# Autodesk Inventor assembly: acrylic kinect bracket - manufacturing
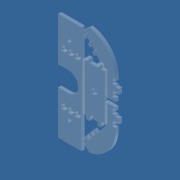
[picture p0: Inventor's stored thumbnail of the model, 180x180]
Saved by Autodesk Inventor 2012 (Build 160160000, 160)
## iProperties
Created: 2012-11-01
Part Number: acrylic kinect bracket - manufacturing
Document SubType Name: Assembly
Designer: Ed
Author: Ed
## Documents named in this file (4)
- C:\Users\Ed\Documents\masters\CAD\Kinect\acrylic kinect bracket - manufacturing.iam
- C:\Users\Ed\Documents\masters\CAD\Kinect\acrylic kinect bracket - bracket.ipt
- C:\Users\Ed\Documents\masters\CAD\Kinect\acrylic kinect bracket - kinect plate.ipt
- C:\Users\Ed\Documents\masters\CAD\Kinect\acrylic kinect plate.ipt
## Components (4 placed, 3 different names)
1. acrylic kinect bracket - bracket:1 — Mate:5, Mate:6, Flush:5, Flush:6
2. acrylic kinect bracket - bracket:2 — Mate:7, Flush:5, Flush:6, Flush:7
3. acrylic kinect bracket - kinect plate:1 — Flush:1, Mate:4, Flush:8
4. acrylic kinect plate:1 — Flush:1, Mate:4, Mate:5, Mate:6, Mate:7, Flush:7, Flush:8
## Relationships (9: Flush 5, Mate 4)
- Flush:1: acrylic kinect bracket - kinect plate:1 ↔ acrylic kinect plate:1
- Mate:4 (2.54 mm): acrylic kinect bracket - kinect plate:1 ↔ acrylic kinect plate:1
- Mate:5 (2.54 mm): acrylic kinect bracket - bracket:1 ↔ acrylic kinect plate:1
- Mate:6: acrylic kinect bracket - bracket:1 ↔ acrylic kinect plate:1
- Mate:7: acrylic kinect bracket - bracket:2 ↔ acrylic kinect plate:1
- Flush:5: acrylic kinect bracket - bracket:1 ↔ acrylic kinect bracket - bracket:2
- Flush:6: acrylic kinect bracket - bracket:1 ↔ acrylic kinect bracket - bracket:2
- Flush:7: acrylic kinect bracket - bracket:2 ↔ acrylic kinect plate:1
- Flush:8 (-63.5 mm): acrylic kinect bracket - kinect plate:1 ↔ acrylic kinect plate:1
